# Autodesk Inventor assembly: body
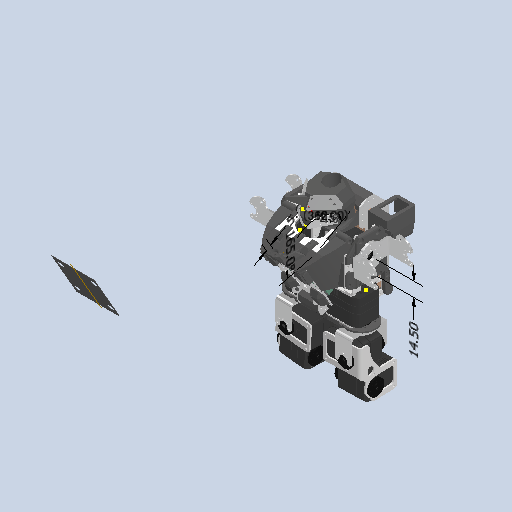
[picture p0: Inventor's stored thumbnail of the model, 512x512]
Saved by Autodesk Inventor 2026.1 (Build 301233020, 233B)
## iProperties
Created: 2024-10-10
Part Number: body
Document SubType Name: Assembly
Designer: hibik
Author: hibik
## Documents named in this file (5)
- C:\Users\hibik\Documents\Robomech\HR\Eglantyne_mark2\hard\body.iam
- C:\Users\hibik\Documents\Robomech\HR\Eglantyne_mark2\hard\under_body\under_body.iam
- C:\Users\hibik\Documents\Robomech\HR\Eglantyne_mark2\hard\upper_body\upperbody.iam
- C:\Users\hibik\Documents\Robomech\HR\Eglantyne_mark2\hard\needed_model\battely.ipt
- C:\Users\hibik\Documents\Robomech\HR\Eglantyne_mark2\hard\head\head.iam
## Components (4 placed, 4 different names)
1. under_body:1 [sub-assembly] — フラッシュ:1, メイト:1, フラッシュ:2
2. battely:1
3. upperbody:1 [sub-assembly] — フラッシュ:1, メイト:1, フラッシュ:2, 挿入:1, 挿入:2
4. head:1 [sub-assembly] — 挿入:1, 挿入:2
## Relationships (5: Flush 2, Insert 2, Mate 1)
- フラッシュ:1 [Flush]: under_body:1 ↔ upperbody:1
- メイト:1 [Mate]: under_body:1 ↔ upperbody:1
- フラッシュ:2 [Flush]: under_body:1 ↔ upperbody:1
- 挿入:1 [Insert]: upperbody:1 ↔ head:1
- 挿入:2 [Insert]: upperbody:1 ↔ head:1
